# Autodesk Inventor assembly: P00173-09-025
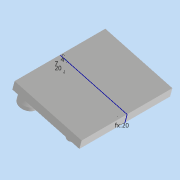
[picture p0: Inventor's stored thumbnail of the model, 180x180]
Saved by Autodesk Inventor 2022 (Build 260153070, 153G)
## iProperties
Created: 2021-08-25
Part Number: P00173-09-025
Document SubType Name: Assembly
Designer: MPM
Author: MPM
Comments: M2-Paypad 3d files for a Cardano blockchain payment terminal. Copyright (C) 2021 Maarten Menheere This program is free software; you can redistribute it and/or modify it under the terms of the GNU General Public License as published by the Free Software Foundation; either version 2 of the License, or (at your option) any later version. This program is distributed in the hope that it will be useful, but WITHOUT ANY WARRANTY; without even the implied warranty of MERCHANTABILITY or FITNESS FOR A PARTICULAR PURPOSE.  See the GNU General Public License for more details. You should have received a copy of the GNU General Public License along with this program; if not, write to the Free Software Foundation, Inc., 51 Franklin Street, Fifth Floor, Boston, MA  02110-1301, USA.
## Documents named in this file (5)
- M:\M2tec\M2tec\P00173 Cashgenic\P00173-09 Paypad - PU Rubber\P00173-09-025.iam
- M:\M2tec\M2tec\P00173 Cashgenic\P00173-09 Paypad - PU Rubber\P00173-09-014.ipt
- M:\M2tec\M2tec\P00173 Cashgenic\P00173-09 Paypad - PU Rubber\P00173-09-012.ipt
- M:\M2tec\M2tec\P00173 Cashgenic\P00173-09 Paypad - PU Rubber\P00173-09-023.ipt
- M:\M2tec\M2tec\P00173 Cashgenic\P00173-09 Paypad - PU Rubber\P00173-09-024.ipt
## Components (16 placed, 4 different names)
1. P00173-09-014:1 — Insert:3, Insert:4, Insert:5, Insert:6, Insert:7, Insert:8, Insert:9, Insert:10, Insert:11, Insert:12, Insert:13, Insert:14, Insert:15, Insert:16, Insert:17
2. P00173-09-023:1 — Insert:5
3. P00173-09-024:1 — Insert:6
4. P00173-09-012:1 — Insert:3
5. P00173-09-012:2 — Insert:4
6. P00173-09-024:2 — Insert:7
7. P00173-09-024:3 — Insert:8
8. P00173-09-024:4 — Insert:9
9. P00173-09-024:5 — Insert:10
10. P00173-09-024:6 — Insert:11
11. P00173-09-023:2 — Insert:12
12. P00173-09-023:3 — Insert:13
13. P00173-09-023:4 — Insert:14
14. P00173-09-023:5 — Insert:15
15. P00173-09-023:6 — Insert:17
16. P00173-09-023:7 — Insert:16
## Relationships (15: Insert 15)
- Insert:3: P00173-09-014:1 ↔ P00173-09-012:1
- Insert:4: P00173-09-014:1 ↔ P00173-09-012:2
- Insert:5: P00173-09-014:1 ↔ P00173-09-023:1
- Insert:6: P00173-09-014:1 ↔ P00173-09-024:1
- Insert:7: P00173-09-014:1 ↔ P00173-09-024:2
- Insert:8: P00173-09-014:1 ↔ P00173-09-024:3
- Insert:9: P00173-09-014:1 ↔ P00173-09-024:4
- Insert:10: P00173-09-014:1 ↔ P00173-09-024:5
- Insert:11: P00173-09-014:1 ↔ P00173-09-024:6
- Insert:12: P00173-09-014:1 ↔ P00173-09-023:2
- Insert:13: P00173-09-014:1 ↔ P00173-09-023:3
- Insert:14: P00173-09-014:1 ↔ P00173-09-023:4
- Insert:15: P00173-09-014:1 ↔ P00173-09-023:5
- Insert:16: P00173-09-014:1 ↔ P00173-09-023:7
- Insert:17: P00173-09-014:1 ↔ P00173-09-023:6
